# Autodesk Inventor assembly: W13-6
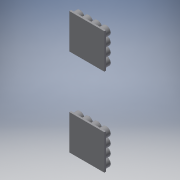
[picture p0: Inventor's stored thumbnail of the model, 180x180]
Saved by Autodesk Inventor 2017 (Build 210142000, 142)
## iProperties
Created: 2020-12-29
Part Number: W13-6
Material: 一般
Document SubType Name: Assembly
Designer: Brian
Sending System: Autodesk Inventor 2020
Preprocessor: ST-DEVELOPER v18
Title: F:\DesktopSpace\MASTERS\ma2010_asm.stp
Author: Crowm
Revision Number: ANY
## Documents named in this file (2)
- E:\coppeliaSim\3D\機械手臂 3D\W13-6.iam
- E:\coppeliaSim\3D\機械手臂 3D\球底座.ipt
## Components (2 placed, 1 different names)
1. 球底座:1 — Flush:3, Flush:4, Mate:33
2. 球底座:2 — Flush:3, Flush:4, Mate:33
## Relationships (3: Flush 2, Mate 1)
- Flush:3: 球底座:1 ↔ 球底座:2
- Flush:4: 球底座:1 ↔ 球底座:2
- Mate:33 (600 mm): 球底座:1 ↔ 球底座:2
